# Autodesk Inventor assembly: ENSAMBLE-COMPLETO
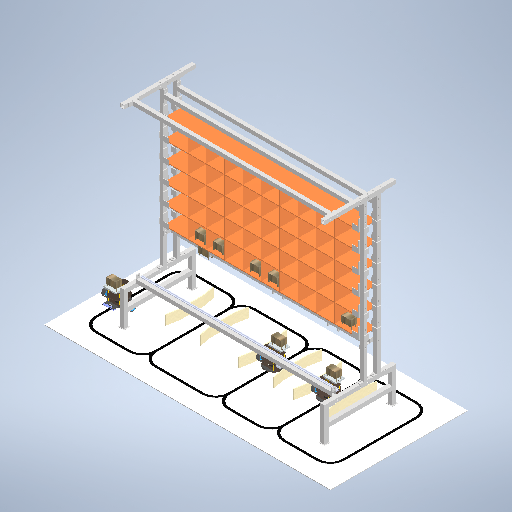
[picture p0: Inventor's stored thumbnail of the model, 512x512]
Saved by Autodesk Inventor 2025.2 (Build 292293000, 293)
## iProperties
Created: 2025-11-05
Part Number: ENSAMBLE-COMPLETO
Document SubType Name: Assembly
Designer: Jonathan Galarza
Author: Jonathan Galarza
## Documents named in this file (10)
- C:\Users\Dax\Documents\Tesis\MODELADO CAD\GARRA\ENSAMBLE-COMPLETO.iam
- C:\Users\Dax\Documents\Tesis\MODELADO CAD\GARRA\Ensamble_STORAGE\Ensamble_STORAGE\Ensamble_STORAGE.ipt
- C:\Users\Dax\Documents\Tesis\MODELADO CAD\GARRA\ENSAMBLE-GARRA.iam
- C:\Users\Dax\Documents\Tesis\MODELADO CAD\Soporte_altura.ipt
- C:\Users\Dax\Documents\Tesis\MODELADO CAD\ARM\ARM.iam
- C:\Users\Dax\Documents\Tesis\MODELADO CAD\tcs230-tcs3200-1.snapshot.1\TCS230-TCS3200\TCS230-TCS3200\TCS230-TCS3200.ipt
- C:\Users\Dax\Documents\Tesis\MODELADO CAD\hw-201-2.snapshot.3\HW-201 v4 90d\HW-201 v4 90d\HW-201 v4 90d.ipt
- C:\Users\Dax\Documents\Tesis\MODELADO CAD\ARM\Caja.ipt
- C:\Users\Dax\Documents\Tesis\MODELADO CAD\pista.ipt
- C:\Users\Dax\Documents\Tesis\MODELADO CAD\guia.ipt
## Components (35 placed, 9 different names)
1. Ensamble_STORAGE:1 — Coincidencia:1, Nivelación:1, Coincidencia:2, Coincidencia:3, Nivelación:2, Coincidencia:4, Coincidencia:5, Nivelación:3, Coincidencia:6, Coincidencia:7, Coincidencia:8, Coincidencia:9, Coincidencia:10, Coincidencia:11, Coincidencia:12, Coincidencia:13, Coincidencia:14, Coincidencia:15, Nivelación:5, Nivelación:6, Nivelación:7, Coincidencia:16, Nivelación:8, Coincidencia:17, Coincidencia:18, Nivelación:9, Coincidencia:19, Coincidencia:20, Nivelación:10, Coincidencia:21, Coincidencia:22, Nivelación:11, Coincidencia:23, Coincidencia:24, Nivelación:12, Coincidencia:25, Coincidencia:26, Nivelación:13, Coincidencia:27, Coincidencia:28, Nivelación:14, Coincidencia:29, Coincidencia:30, Nivelación:15, Coincidencia:31, Coincidencia:32, Nivelación:16, Coincidencia:33, Coincidencia:34, Nivelación:17, Coincidencia:35, Coincidencia:36, Coincidencia:37, Coincidencia:38, Coincidencia:39, Coincidencia:40, Nivelación:18, Nivelación:19, Nivelación:20, Nivelación:21, Nivelación:22, Coincidencia:41, Coincidencia:42, Coincidencia:43, Coincidencia:44, Coincidencia:45, Nivelación:27, Nivelación:28, Nivelación:29, Coincidencia:64, Coincidencia:65, Coincidencia:66, Coincidencia:67, Coincidencia:68, Coincidencia:69
2. ENSAMBLE-GARRA:1 [sub-assembly] — Coincidencia:1, Nivelación:1, Coincidencia:2, Coincidencia:48
3. ENSAMBLE-GARRA:2 [sub-assembly] — Coincidencia:3, Nivelación:2, Coincidencia:4, Coincidencia:47
4. ENSAMBLE-GARRA:3 [sub-assembly] — Coincidencia:5, Nivelación:3, Coincidencia:6, Coincidencia:49, Nivelación:25, Nivelación:26
5. Soporte_altura:1 — Coincidencia:10, Coincidencia:11, Coincidencia:12, Nivelación:4, Nivelación:24, Coincidencia:50, Nivelación:30, Nivelación:31
6. Soporte_altura:2 — Coincidencia:7, Coincidencia:8, Coincidencia:9
7. ARM:1 [sub-assembly] — Nivelación:4, Coincidencia:47
8. TCS230-TCS3200:1 — Coincidencia:13, Nivelación:7, Nivelación:27
9. TCS230-TCS3200:2 — Coincidencia:14, Nivelación:6, Nivelación:28
10. TCS230-TCS3200:3 — Coincidencia:15, Nivelación:5, Nivelación:29
11. HW-201 v4 90d:1 — Coincidencia:16, Nivelación:8, Coincidencia:17
12. HW-201 v4 90d:2 — Coincidencia:18, Nivelación:9, Coincidencia:19
13. HW-201 v4 90d:3 — Coincidencia:20, Nivelación:10, Coincidencia:21
14. HW-201 v4 90d:4 — Coincidencia:22, Nivelación:11, Coincidencia:23
15. HW-201 v4 90d:5 — Coincidencia:24, Nivelación:12, Coincidencia:25
16. HW-201 v4 90d:6 — Coincidencia:26, Nivelación:13, Coincidencia:27
17. HW-201 v4 90d:7 — Coincidencia:28, Nivelación:14, Coincidencia:29
18. HW-201 v4 90d:8 — Coincidencia:30, Nivelación:15, Coincidencia:31
19. HW-201 v4 90d:9 — Coincidencia:32, Nivelación:16, Coincidencia:33
20. HW-201 v4 90d:10 — Coincidencia:34, Nivelación:17, Coincidencia:35
21. Caja:1 — Coincidencia:37, Nivelación:18, Coincidencia:41
22. Caja:2 — Coincidencia:36, Nivelación:19, Coincidencia:42
23. Caja:3 — Coincidencia:38, Nivelación:20, Coincidencia:43
24. Caja:4 — Coincidencia:39, Nivelación:21, Coincidencia:44
25. Caja:5 — Coincidencia:40, Nivelación:22, Coincidencia:45
26. ARM:2 [sub-assembly] — Nivelación:24, Coincidencia:48
27. Caja:6 — Coincidencia:49, Nivelación:25, Nivelación:26
28. pista:1 — Coincidencia:50, Nivelación:30, Nivelación:31, Coincidencia:51, Coincidencia:52, Coincidencia:53, Coincidencia:54, Coincidencia:55, Coincidencia:56, Coincidencia:57, Coincidencia:58, Coincidencia:59, Coincidencia:60, Coincidencia:61, Coincidencia:62, Coincidencia:63
29. ARM:5 [sub-assembly] — Coincidencia:51
30. guia:1 — Coincidencia:52, Coincidencia:53, Coincidencia:64
31. guia:2 — Coincidencia:56, Coincidencia:57, Coincidencia:65
32. guia:3 — Coincidencia:60, Coincidencia:61, Coincidencia:66
33. guia:4 — Coincidencia:62, Coincidencia:63, Coincidencia:69
34. guia:5 — Coincidencia:58, Coincidencia:59, Coincidencia:68
35. guia:6 — Coincidencia:54, Coincidencia:55, Coincidencia:67
## Relationships (98: Mate 68, Flush 30)
- Coincidencia:1 [Mate]: Ensamble_STORAGE:1 ↔ ENSAMBLE-GARRA:1
- Nivelación:1 [Flush]: Ensamble_STORAGE:1 ↔ ENSAMBLE-GARRA:1
- Coincidencia:2 [Mate] (32.5 mm): Ensamble_STORAGE:1 ↔ ENSAMBLE-GARRA:1
- Coincidencia:3 [Mate]: Ensamble_STORAGE:1 ↔ ENSAMBLE-GARRA:2
- Nivelación:2 [Flush]: Ensamble_STORAGE:1 ↔ ENSAMBLE-GARRA:2
- Coincidencia:4 [Mate] (32.5 mm): Ensamble_STORAGE:1 ↔ ENSAMBLE-GARRA:2
- Coincidencia:5 [Mate]: Ensamble_STORAGE:1 ↔ ENSAMBLE-GARRA:3
- Nivelación:3 [Flush]: Ensamble_STORAGE:1 ↔ ENSAMBLE-GARRA:3
- Coincidencia:6 [Mate] (32.5 mm): Ensamble_STORAGE:1 ↔ ENSAMBLE-GARRA:3
- Coincidencia:7 [Mate]: Ensamble_STORAGE:1 ↔ Soporte_altura:2
- Coincidencia:8 [Mate]: Ensamble_STORAGE:1 ↔ Soporte_altura:2
- Coincidencia:9 [Mate]: Ensamble_STORAGE:1 ↔ Soporte_altura:2
- Coincidencia:10 [Mate]: Ensamble_STORAGE:1 ↔ Soporte_altura:1
- Coincidencia:11 [Mate]: Ensamble_STORAGE:1 ↔ Soporte_altura:1
- Coincidencia:12 [Mate]: Ensamble_STORAGE:1 ↔ Soporte_altura:1
- Nivelación:4 [Flush] (18 mm): Soporte_altura:1 ↔ ARM:1
- Coincidencia:13 [Mate]: Ensamble_STORAGE:1 ↔ TCS230-TCS3200:1
- Coincidencia:14 [Mate]: Ensamble_STORAGE:1 ↔ TCS230-TCS3200:2
- Coincidencia:15 [Mate]: Ensamble_STORAGE:1 ↔ TCS230-TCS3200:3
- Nivelación:5 [Flush] (65 mm): Ensamble_STORAGE:1 ↔ TCS230-TCS3200:3
- Nivelación:6 [Flush] (65 mm): Ensamble_STORAGE:1 ↔ TCS230-TCS3200:2
- Nivelación:7 [Flush] (65 mm): Ensamble_STORAGE:1 ↔ TCS230-TCS3200:1
- Coincidencia:16 [Mate]: Ensamble_STORAGE:1 ↔ HW-201 v4 90d:1
- Nivelación:8 [Flush] (30 mm): Ensamble_STORAGE:1 ↔ HW-201 v4 90d:1
- Coincidencia:17 [Mate] (70 mm): Ensamble_STORAGE:1 ↔ HW-201 v4 90d:1
- Coincidencia:18 [Mate]: Ensamble_STORAGE:1 ↔ HW-201 v4 90d:2
- Nivelación:9 [Flush] (30 mm): Ensamble_STORAGE:1 ↔ HW-201 v4 90d:2
- Coincidencia:19 [Mate] (70 mm): Ensamble_STORAGE:1 ↔ HW-201 v4 90d:2
- Coincidencia:20 [Mate]: Ensamble_STORAGE:1 ↔ HW-201 v4 90d:3
- Nivelación:10 [Flush] (30 mm): Ensamble_STORAGE:1 ↔ HW-201 v4 90d:3
- Coincidencia:21 [Mate] (70 mm): Ensamble_STORAGE:1 ↔ HW-201 v4 90d:3
- Coincidencia:22 [Mate]: Ensamble_STORAGE:1 ↔ HW-201 v4 90d:4
- Nivelación:11 [Flush] (30 mm): Ensamble_STORAGE:1 ↔ HW-201 v4 90d:4
- Coincidencia:23 [Mate] (70 mm): Ensamble_STORAGE:1 ↔ HW-201 v4 90d:4
- Coincidencia:24 [Mate]: Ensamble_STORAGE:1 ↔ HW-201 v4 90d:5
- Nivelación:12 [Flush] (30 mm): Ensamble_STORAGE:1 ↔ HW-201 v4 90d:5
- Coincidencia:25 [Mate] (70 mm): Ensamble_STORAGE:1 ↔ HW-201 v4 90d:5
- Coincidencia:26 [Mate]: Ensamble_STORAGE:1 ↔ HW-201 v4 90d:6
- Nivelación:13 [Flush] (30 mm): Ensamble_STORAGE:1 ↔ HW-201 v4 90d:6
- Coincidencia:27 [Mate] (70 mm): Ensamble_STORAGE:1 ↔ HW-201 v4 90d:6
- Coincidencia:28 [Mate]: Ensamble_STORAGE:1 ↔ HW-201 v4 90d:7
- Nivelación:14 [Flush] (30 mm): Ensamble_STORAGE:1 ↔ HW-201 v4 90d:7
- Coincidencia:29 [Mate] (70 mm): Ensamble_STORAGE:1 ↔ HW-201 v4 90d:7
- Coincidencia:30 [Mate]: Ensamble_STORAGE:1 ↔ HW-201 v4 90d:8
- Nivelación:15 [Flush] (30 mm): Ensamble_STORAGE:1 ↔ HW-201 v4 90d:8
- Coincidencia:31 [Mate] (70 mm): Ensamble_STORAGE:1 ↔ HW-201 v4 90d:8
- Coincidencia:32 [Mate]: Ensamble_STORAGE:1 ↔ HW-201 v4 90d:9
- Nivelación:16 [Flush] (30 mm): Ensamble_STORAGE:1 ↔ HW-201 v4 90d:9
- Coincidencia:33 [Mate] (70 mm): Ensamble_STORAGE:1 ↔ HW-201 v4 90d:9
- Coincidencia:34 [Mate]: Ensamble_STORAGE:1 ↔ HW-201 v4 90d:10
- Nivelación:17 [Flush] (30 mm): Ensamble_STORAGE:1 ↔ HW-201 v4 90d:10
- Coincidencia:35 [Mate] (70 mm): Ensamble_STORAGE:1 ↔ HW-201 v4 90d:10
- Coincidencia:36 [Mate]: Ensamble_STORAGE:1 ↔ Caja:2
- Coincidencia:37 [Mate]: Ensamble_STORAGE:1 ↔ Caja:1
- Coincidencia:38 [Mate]: Ensamble_STORAGE:1 ↔ Caja:3
- Coincidencia:39 [Mate]: Ensamble_STORAGE:1 ↔ Caja:4
- Coincidencia:40 [Mate]: Ensamble_STORAGE:1 ↔ Caja:5
- Nivelación:18 [Flush] (20 mm): Ensamble_STORAGE:1 ↔ Caja:1
- Nivelación:19 [Flush] (20 mm): Ensamble_STORAGE:1 ↔ Caja:2
- Nivelación:20 [Flush] (20 mm): Ensamble_STORAGE:1 ↔ Caja:3
- Nivelación:21 [Flush] (20 mm): Ensamble_STORAGE:1 ↔ Caja:4
- Nivelación:22 [Flush] (20 mm): Ensamble_STORAGE:1 ↔ Caja:5
- Coincidencia:41 [Mate] (35 mm): Ensamble_STORAGE:1 ↔ Caja:1
- Coincidencia:42 [Mate] (35 mm): Ensamble_STORAGE:1 ↔ Caja:2
- Coincidencia:43 [Mate] (35 mm): Ensamble_STORAGE:1 ↔ Caja:3
- Coincidencia:44 [Mate] (35 mm): Ensamble_STORAGE:1 ↔ Caja:4
- Coincidencia:45 [Mate] (35 mm): Ensamble_STORAGE:1 ↔ Caja:5
- Nivelación:24 [Flush] (18 mm): Soporte_altura:1 ↔ ARM:2
- Coincidencia:47 [Mate] (10 mm): ENSAMBLE-GARRA:2 ↔ ARM:1
- Coincidencia:48 [Mate] (10 mm): ENSAMBLE-GARRA:1 ↔ ARM:2
- Coincidencia:49 [Mate]: ENSAMBLE-GARRA:3 ↔ Caja:6
- Nivelación:25 [Flush]: ENSAMBLE-GARRA:3 ↔ Caja:6
- Nivelación:26 [Flush] (-5 mm): ENSAMBLE-GARRA:3 ↔ Caja:6
- Nivelación:27 [Flush] (5 mm): Ensamble_STORAGE:1 ↔ TCS230-TCS3200:1
- Nivelación:28 [Flush] (5 mm): Ensamble_STORAGE:1 ↔ TCS230-TCS3200:2
- Nivelación:29 [Flush] (5 mm): Ensamble_STORAGE:1 ↔ TCS230-TCS3200:3
- Coincidencia:50 [Mate]: Soporte_altura:1 ↔ pista:1
- Nivelación:30 [Flush] (-300 mm): Soporte_altura:1 ↔ pista:1
- Nivelación:31 [Flush] (-350 mm): Soporte_altura:1 ↔ pista:1
- Coincidencia:51 [Mate] (18 mm): pista:1 ↔ ARM:5
- Coincidencia:52 [Mate]: pista:1 ↔ guia:1
- Coincidencia:53 [Mate] (115 mm): pista:1 ↔ guia:1
- Coincidencia:54 [Mate]: pista:1 ↔ guia:6
- Coincidencia:55 [Mate] (115 mm): pista:1 ↔ guia:6
- Coincidencia:56 [Mate]: pista:1 ↔ guia:2
- Coincidencia:57 [Mate] (115 mm): pista:1 ↔ guia:2
- Coincidencia:58 [Mate]: pista:1 ↔ guia:5
- Coincidencia:59 [Mate] (115 mm): pista:1 ↔ guia:5
- Coincidencia:60 [Mate]: pista:1 ↔ guia:3
- Coincidencia:61 [Mate] (115 mm): pista:1 ↔ guia:3
- Coincidencia:62 [Mate]: pista:1 ↔ guia:4
- Coincidencia:63 [Mate] (115 mm): pista:1 ↔ guia:4
- Coincidencia:64 [Mate] (25 mm): Ensamble_STORAGE:1 ↔ guia:1
- Coincidencia:65 [Mate] (25 mm): Ensamble_STORAGE:1 ↔ guia:2
- Coincidencia:66 [Mate] (25 mm): Ensamble_STORAGE:1 ↔ guia:3
- Coincidencia:67 [Mate] (25 mm): Ensamble_STORAGE:1 ↔ guia:6
- Coincidencia:68 [Mate] (25 mm): Ensamble_STORAGE:1 ↔ guia:5
- Coincidencia:69 [Mate] (25 mm): Ensamble_STORAGE:1 ↔ guia:4
